# Autodesk Inventor assembly: wooden
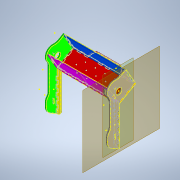
[picture p0: Inventor's stored thumbnail of the model, 180x180]
Saved by Autodesk Inventor 2020 (Build 240168000, 168)
## iProperties
Created: 2019-07-24
Part Number: wooden
Document SubType Name: Assembly
Designer: erwin
Author: erwin
## Documents named in this file (7)
- D:\GitHub\BeachMaid\platform\wooden_assembly.iam
- D:\GitHub\BeachMaid\platform\wooden_side.ipt
- D:\GitHub\BeachMaid\platform\wooden_lip.ipt
- D:\GitHub\BeachMaid\platform\wooden_back.ipt
- D:\GitHub\BeachMaid\platform\dxf\wooden_bottom.ipt
- D:\GitHub\BeachMaid\platform\wooden_top.ipt
- D:\GitHub\BeachMaid\platform\wooden_stiffener.ipt
## Components (8 placed, 6 different names)
1. wooden_side:1 — Flush:1, Flush:2, Flush:3, Flush:4, Flush:5, Flush:6, Flush:7, Flush:8, Flush:9, Flush:10, Flush:11, Flush:12, Flush:20, Flush:21
2. wooden_lip:1 — Flush:1, Flush:2, Flush:3
3. wooden_back:1 — Flush:4, Flush:5, Flush:6, Flush:7, Flush:14, Flush:16, Flush:17, Mate:1, Mate:2, Mate:3
4. wooden_bottom:1 — Flush:8, Flush:9, Flush:10, Flush:11, Flush:12, Flush:15
5. wooden_side:2 — Flush:14, Flush:15, Flush:18, Mate:4, Flush:19
6. wooden_top:1 — Flush:16, Flush:17, Mate:1, Mate:2, Mate:3
7. wooden_lip:2 — Flush:18, Mate:4, Flush:19
8. wooden_stiffener:1 — Flush:20, Flush:21
## Relationships (24: Flush 20, Mate 4)
- Flush:1: wooden_side:1 ↔ wooden_lip:1
- Flush:2: wooden_side:1 ↔ wooden_lip:1
- Flush:3: wooden_side:1 ↔ wooden_lip:1
- Flush:4: wooden_side:1 ↔ wooden_back:1
- Flush:5: wooden_side:1 ↔ wooden_back:1
- Flush:6: wooden_side:1 ↔ wooden_back:1
- Flush:7: wooden_side:1 ↔ wooden_back:1
- Flush:8: wooden_side:1 ↔ wooden_bottom:1
- Flush:9: wooden_side:1 ↔ wooden_bottom:1
- Flush:10: wooden_side:1 ↔ wooden_bottom:1
- Flush:11: wooden_side:1 ↔ wooden_bottom:1
- Flush:12: wooden_side:1 ↔ wooden_bottom:1
- Flush:14: wooden_back:1 ↔ wooden_side:2
- Flush:15: wooden_bottom:1 ↔ wooden_side:2
- Flush:16: wooden_back:1 ↔ wooden_top:1
- Flush:17: wooden_back:1 ↔ wooden_top:1
- Mate:1: wooden_back:1 ↔ wooden_top:1
- Mate:2: wooden_back:1 ↔ wooden_top:1
- Mate:3: wooden_back:1 ↔ wooden_top:1
- Flush:18: wooden_side:2 ↔ wooden_lip:2
- Mate:4: wooden_side:2 ↔ wooden_lip:2
- Flush:19: wooden_side:2 ↔ wooden_lip:2
- Flush:20: wooden_side:1 ↔ wooden_stiffener:1
- Flush:21 (20 mm): wooden_side:1 ↔ wooden_stiffener:1
